# Autodesk Inventor assembly: Robot
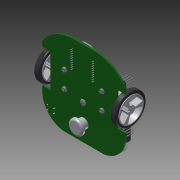
[picture p0: Inventor's stored thumbnail of the model, 180x180]
Saved by Autodesk Inventor 2014 SP2 (Build 180246200, 246)
## iProperties
Created: 2015-03-17
Part Number: Robot
Document SubType Name: Assembly
Designer: sd
Author: sd
## Documents named in this file (15)
- D:\Utilisateurs\sd\Mes documents\SVN\projets-gei\Dumber 2015\Mecanique\Robot.iam
- D:\Utilisateurs\sd\Mes documents\SVN\projets-gei\Dumber 2015\Mecanique\pcb.ipt
- D:\Utilisateurs\sd\Mes documents\SVN\projets-gei\Dumber 2015\Mecanique\Bloc roue.iam
- D:\Utilisateurs\sd\Mes documents\Inventor\Content Center Files\R2014\fr-FR\GB_T 2671.1-2004\Screw GB_T 2171.1 M2,5 x 5.ipt
- D:\Utilisateurs\sd\Mes documents\Inventor\Content Center Files\R2014\fr-FR\ISO 4035(2)\ISO 4035 - M2,5ISO.ipt
- D:\Utilisateurs\sd\Mes documents\SVN\projets-gei\Dumber 2015\Mecanique\Batterie.ipt
- D:\Utilisateurs\sd\Mes documents\SVN\projets-gei\Dumber 2015\Mecanique\connecteur 6.ipt
- D:\Utilisateurs\sd\Mes documents\SVN\projets-gei\Dumber 2015\Mecanique\pied.ipt
- D:\Utilisateurs\sd\Mes documents\Inventor\Content Center Files\R2014\fr-FR\GB_T 2671.1-2004\Screw GB_T 2171.1 M3 x 8.ipt
- D:\Utilisateurs\sd\Mes documents\SVN\projets-gei\Dumber 2015\Mecanique\Composants importés\USB_Mini_B_SMD_buchse\USB_Mini_B_SMD_buchse.ipt
- D:\Utilisateurs\sd\Mes documents\SVN\projets-gei\Dumber 2015\Mecanique\Composants importés\tactileswitch-short\tactileswitch-short.ipt
- D:\Utilisateurs\sd\Mes documents\SVN\projets-gei\Dumber 2015\Mecanique\Composants importés\XBee Chip\XBee Chip.iam
- D:\Utilisateurs\sd\Mes documents\SVN\projets-gei\Dumber 2015\Mecanique\Composants importés\0605-LED_Verde\0605-LED_Verde.ipt
- D:\Utilisateurs\sd\Mes documents\SVN\projets-gei\Dumber 2015\Mecanique\capot.ipt
- D:\Utilisateurs\sd\Mes documents\Inventor\Content Center Files\R2014\fr-FR\GB_T 2671.1-2004\Screw GB_T 2171.1 M2,5 x 6.ipt
## Components (28 placed, 14 different names)
1. pcb:1 — Placage:1, Placage:2, Placage:3, Placage:4, Placage:5, Placage:6, Logement:1, Logement:2, Logement:3, Logement:4, Placage:12, Angle:1, Placage:13, Placage:15, Placage:16, Placage:17, Angle:2, Angle:4, Placage:18, Placage:19, Placage:20, Angle:8, Angle:9, Placage:22, Placage:23, Angle:10, Angle:11, Placage:24, Placage:25, Placage:26, Angle:12, Placage:27, Placage:28, Placage:29, Angle:13, Placage:30, Logement:7
2. Bloc roue:1 [sub-assembly] — Placage:2, Placage:3, Placage:4
3. Bloc roue:2 [sub-assembly] — Placage:1, Placage:5, Placage:6
4. Screw GB/T 2671.1-2004 M2.5x5 Property Class 4.8:1 — Logement:1, Placage:7, Placage:8
5. Screw GB/T 2671.1-2004 M2.5x5 Property Class 4.8:2 — Logement:2, Placage:11
6. Screw GB/T 2671.1-2004 M2.5x5 Property Class 4.8:3 — Logement:3, Placage:9
7. Screw GB/T 2671.1-2004 M2.5x5 Property Class 4.8:4 — Logement:4, Placage:10
8. ISO 4035 M2,5:1 — Placage:7, Placage:8
9. ISO 4035 M2,5:2 — Placage:10
10. ISO 4035 M2,5:3 — Placage:9
11. ISO 4035 M2,5:4 — Placage:11
12. Batterie:1 — Placage:12, Angle:1, Placage:18, Logement:5
13. connecteur 6:1 — Placage:15, Angle:8
14. connecteur 6:2 — Placage:13, Angle:2
15. connecteur 6:3 — Placage:16, Angle:4
16. connecteur 6:4 — Placage:17, Angle:9
17. pied:1 — Placage:19, Placage:20
18. Screw GB/T 2671.1-2004 M3x8 Property Class 4.8:1 — Logement:5
19. connecteur 6:5 — Placage:22, Angle:10
20. connecteur 6:6 — Placage:23, Angle:11
21. USB_Mini_B_SMD_buchse:1 — Placage:24
22. tactileswitch-short:1 — Placage:25
23. XBee Chip:1 [sub-assembly] — Placage:26, Angle:12
24. 0605-LED_Verde:1 — Placage:27
25. 0605-LED_Verde:2 — Placage:28
26. capot:1 — Placage:29, Angle:13, Placage:30, Logement:6
27. Screw GB/T 2671.1-2004 M2.5x6 Property Class 4.8:1 — Logement:6
28. ISO 4035 M2,5:5 — Logement:7
## Relationships (44: Mate 28, Angle 9, Insert 7)
- Placage:1 [Mate]: pcb:1 ↔ Bloc roue:2
- Placage:2 [Mate]: pcb:1 ↔ Bloc roue:1
- Placage:3 [Mate]: pcb:1 ↔ Bloc roue:1
- Placage:4 [Mate]: pcb:1 ↔ Bloc roue:1
- Placage:5 [Mate]: pcb:1 ↔ Bloc roue:2
- Placage:6 [Mate]: pcb:1 ↔ Bloc roue:2
- Logement:1 [Insert]: pcb:1 ↔ Screw GB/T 2671.1-2004 M2.5x5 Property Class 4.8:1
- Logement:2 [Insert]: pcb:1 ↔ Screw GB/T 2671.1-2004 M2.5x5 Property Class 4.8:2
- Logement:3 [Insert]: pcb:1 ↔ Screw GB/T 2671.1-2004 M2.5x5 Property Class 4.8:3
- Logement:4 [Insert]: pcb:1 ↔ Screw GB/T 2671.1-2004 M2.5x5 Property Class 4.8:4
- Placage:7 [Mate]: Screw GB/T 2671.1-2004 M2.5x5 Property Class 4.8:1 ↔ ISO 4035 M2,5:1
- Placage:8 [Mate] (-1.5 mm): Screw GB/T 2671.1-2004 M2.5x5 Property Class 4.8:1 ↔ ISO 4035 M2,5:1
- Placage:9 [Mate]: Screw GB/T 2671.1-2004 M2.5x5 Property Class 4.8:3 ↔ ISO 4035 M2,5:3
- Placage:10 [Mate]: Screw GB/T 2671.1-2004 M2.5x5 Property Class 4.8:4 ↔ ISO 4035 M2,5:2
- Placage:11 [Mate]: Screw GB/T 2671.1-2004 M2.5x5 Property Class 4.8:2 ↔ ISO 4035 M2,5:4
- Placage:12 [Mate]: pcb:1 ↔ Batterie:1
- Angle:1 (0 deg): pcb:1 ↔ Batterie:1
- Placage:13 [Mate]: pcb:1 ↔ connecteur 6:2
- Placage:15 [Mate]: pcb:1 ↔ connecteur 6:1
- Placage:16 [Mate]: pcb:1 ↔ connecteur 6:3
- Placage:17 [Mate]: pcb:1 ↔ connecteur 6:4
- Angle:2 (0 deg): pcb:1 ↔ connecteur 6:2
- Angle:4 (0 deg): pcb:1 ↔ connecteur 6:3
- Placage:18 [Mate]: pcb:1 ↔ Batterie:1
- Placage:19 [Mate]: pcb:1 ↔ pied:1
- Placage:20 [Mate]: pcb:1 ↔ pied:1
- Logement:5 [Insert]: Batterie:1 ↔ Screw GB/T 2671.1-2004 M3x8 Property Class 4.8:1
- Angle:8 (0 deg): pcb:1 ↔ connecteur 6:1
- Angle:9 (0 deg): pcb:1 ↔ connecteur 6:4
- Placage:22 [Mate]: pcb:1 ↔ connecteur 6:5
- Placage:23 [Mate]: pcb:1 ↔ connecteur 6:6
- Angle:10 (0 deg): pcb:1 ↔ connecteur 6:5
- Angle:11 (0 deg): pcb:1 ↔ connecteur 6:6
- Placage:24 [Mate]: pcb:1 ↔ USB_Mini_B_SMD_buchse:1
- Placage:25 [Mate]: pcb:1 ↔ tactileswitch-short:1
- Placage:26 [Mate]: pcb:1 ↔ XBee Chip:1
- Angle:12 (0 deg): pcb:1 ↔ XBee Chip:1
- Placage:27 [Mate]: pcb:1 ↔ 0605-LED_Verde:1
- Placage:28 [Mate]: pcb:1 ↔ 0605-LED_Verde:2
- Placage:29 [Mate]: pcb:1 ↔ capot:1
- Angle:13 (0 deg): pcb:1 ↔ capot:1
- Placage:30 [Mate]: pcb:1 ↔ capot:1
- Logement:6 [Insert]: capot:1 ↔ Screw GB/T 2671.1-2004 M2.5x6 Property Class 4.8:1
- Logement:7 [Insert]: pcb:1 ↔ ISO 4035 M2,5:5
